# Autodesk Inventor assembly: sestav mehanizma
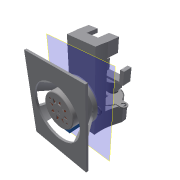
[picture p0: Inventor's stored thumbnail of the model, 180x180]
Saved by Autodesk Inventor 2018.3 (Build 223284000, 284)
## iProperties
Created: 2020-03-05
Part Number: sestav mehanizma
Document SubType Name: Assembly
Designer: Erik
Author: Erik
## Documents named in this file (5)
- D:\DUsers\Documents\Inventor\Projekti 2020\AVMS - 3D skener\prototipV01\sestav mehanizma.iam
- D:\DUsers\Documents\Inventor\Projekti 2020\AVMS - 3D skener\Non printed\sensor holder.ipt
- D:\DUsers\Documents\Inventor\Projekti 2020\AVMS - 3D skener\Non printed\28BYJ-48-stepper.ipt
- D:\DUsers\Documents\Inventor\Projekti 2020\AVMS - 3D skener\prototipV01\segment_1.ipt
- D:\DUsers\Documents\Inventor\Projekti 2020\AVMS - 3D skener\prototipV01\Base.ipt
## Components (5 placed, 4 different names)
1. sensor holder:1 — Rotational:1, Mate:1
2. 28BYJ-48-stepper:1 — Rotational:1, Angle:1, Mate:2, Angle:2
3. 28BYJ-48-stepper:2 — Angle:1, Mate:1, Mate:2, Angle:2, Flush:1, Flush:2
4. segment_1:1 — Flush:1
5. Base:1 — Flush:2
## Relationships (7: Angle 2, Mate 2, Flush 2, RevoluteJoint 1)
- Rotational:1 [RevoluteJoint]: sensor holder:1 ↔ 28BYJ-48-stepper:1
- Angle:1 (180 deg): 28BYJ-48-stepper:1 ↔ 28BYJ-48-stepper:2
- Mate:1: sensor holder:1 ↔ 28BYJ-48-stepper:2
- Mate:2 (10 mm): 28BYJ-48-stepper:1 ↔ 28BYJ-48-stepper:2
- Angle:2 (0 deg): 28BYJ-48-stepper:1 ↔ 28BYJ-48-stepper:2
- Flush:1: 28BYJ-48-stepper:2 ↔ segment_1:1
- Flush:2: 28BYJ-48-stepper:2 ↔ Base:1
